# Autodesk Inventor assembly: MTLV-S05
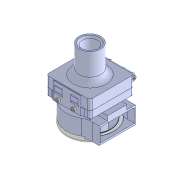
[picture p0: Inventor's stored thumbnail of the model, 180x180]
Saved by Autodesk Inventor 2020 (Build 240168000, 168)
## iProperties
Created: 2020-03-28
Part Number: MTLV-S05
Document SubType Name: Assembly
Designer: John K
Author: John K
## Documents named in this file (8)
- C:\GrabCAD\MTL Ventilator Design\MTLV\Subassemblies\MTLV-S05.iam
- C:\GrabCAD\MTL Ventilator Design\MTLV\Manufactured Parts\MTLV-P06.ipt
- C:\GrabCAD\MTL Ventilator Design\MTLV\Manufactured Parts\MTLV-P04.ipt
- C:\GrabCAD\MTL Ventilator Design\MTLV\Manufactured Parts\MTLV-P05.ipt
- C:\GrabCAD\MTL Ventilator Design\MTLV\Manufactured Parts\MTLV-P07.ipt
- C:\GrabCAD\MTL Ventilator Design\MTLV\Commercial Parts\Fasteners\M3x10mm Socket.ipt
- C:\GrabCAD\MTL Ventilator Design\MTLV\Commercial Parts\Fasteners\M4x40mm Socket.ipt
- C:\GrabCAD\MTL Ventilator Design\MTLV\Manufactured Parts\MTLV-M09.ipt
## Components (12 placed, 7 different names)
1. MTLV-P06:1 — Mate:1, Flush:1, Mate:2, Mate:3, Mate:4, Mate:5, Mate:6, Insert:1, Mate:7, Insert:4, Insert:5, Insert:6, Insert:7
2. MTLV-P04:1 — Mate:1, Flush:1, Mate:2, Insert:8
3. MTLV-P05:1 — Mate:3, Mate:4, Mate:5, Insert:2, Insert:3
4. MTLV-P07:1 — Mate:6, Mate:7
5. MTLV-M09:1 — Insert:1
6. M3x10mm Socket:1 — Insert:2
7. M3x10mm Socket:2 — Insert:3
8. M3x10mm Socket:3 — Insert:4
9. M3x10mm Socket:4 — Insert:5
10. M3x10mm Socket:5 — Insert:6
11. M3x10mm Socket:6 — Insert:7
12. M4x40mm Socket:1 — Insert:8
## Relationships (16: Insert 8, Mate 7, Flush 1)
- Mate:1: MTLV-P06:1 ↔ MTLV-P04:1
- Flush:1: MTLV-P06:1 ↔ MTLV-P04:1
- Mate:2: MTLV-P06:1 ↔ MTLV-P04:1
- Mate:3: MTLV-P06:1 ↔ MTLV-P05:1
- Mate:4: MTLV-P06:1 ↔ MTLV-P05:1
- Mate:5: MTLV-P06:1 ↔ MTLV-P05:1
- Mate:6: MTLV-P06:1 ↔ MTLV-P07:1
- Insert:1: MTLV-P06:1 ↔ MTLV-M09:1
- Mate:7: MTLV-P06:1 ↔ MTLV-P07:1
- Insert:2: MTLV-P05:1 ↔ M3x10mm Socket:1
- Insert:3: MTLV-P05:1 ↔ M3x10mm Socket:2
- Insert:4: MTLV-P06:1 ↔ M3x10mm Socket:3
- Insert:5: MTLV-P06:1 ↔ M3x10mm Socket:4
- Insert:6: MTLV-P06:1 ↔ M3x10mm Socket:5
- Insert:7: MTLV-P06:1 ↔ M3x10mm Socket:6
- Insert:8: MTLV-P04:1 ↔ M4x40mm Socket:1
